# Autodesk Inventor assembly: lower arm full Assembly 800.ipt
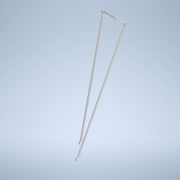
[picture p0: Inventor's stored thumbnail of the model, 180x180]
Saved by Autodesk Inventor 2021 (Build 250183000, 183)
## iProperties
Created: 2022-09-08
Part Number: lower arm full Assembly 800.ipt
Document SubType Name: Assembly
Designer: Administrator
Title: lower arm
Author: Administrator
## Documents named in this file (6)
- C:\Users\szucs\Desktop\GTPR\ver2\lower arm full Assembly 800.ipt.iam
- C:\Users\szucs\Desktop\GTPR\ver2\elbow keeper v1.ipt
- C:\Users\szucs\Desktop\GTPR\ver2\washer v1.ipt
- C:\Users\szucs\Desktop\GTPR\ver2\M8 Nut v5 v1.ipt
- C:\Users\szucs\Desktop\GTPR\ver2\lower arm Assembly 800.ipt.iam
- lower arm Assembly 800.ipt
## Components (13 placed, 4 different names)
1. elbow keeper v1:1 — Mate:1, Mate:3, Mate:6, Mate:7
2. washer v1:1 — Mate:2
3. washer v1:2 — Mate:9, Mate:10
4. washer v1:3 — Mate:8
5. washer v1:4 — Mate:4
6. M8 Nut v5 v1:1
7. M8 Nut v5 v1:2 — Flush:2
8. M8 Nut v5 v1:3 — Flush:1, Mate:10
9. M8 Nut v5 v1:4
10. lower arm Assembly 800.ipt:1 [sub-assembly] — Mate:1, Mate:2, Mate:9
11. lower arm Assembly 800.ipt:2 [sub-assembly] — Mate:3, Mate:4, Mate:8
12. M8 Nut v5 v1:5 — Flush:2, Mate:7
13. M8 Nut v5 v1:6 — Flush:1, Mate:6
## Relationships (11: Mate 9, Flush 2)
- Mate:1: elbow keeper v1:1 ↔ lower arm Assembly 800.ipt:1
- Mate:2: washer v1:1 ↔ lower arm Assembly 800.ipt:1
- Mate:3: elbow keeper v1:1 ↔ lower arm Assembly 800.ipt:2
- Mate:4: washer v1:4 ↔ lower arm Assembly 800.ipt:2
- Flush:1 (-22.5 mm): M8 Nut v5 v1:3 ↔ M8 Nut v5 v1:6
- Mate:6: elbow keeper v1:1 ↔ M8 Nut v5 v1:6
- Flush:2 (-22.5 mm): M8 Nut v5 v1:2 ↔ M8 Nut v5 v1:5
- Mate:7: elbow keeper v1:1 ↔ M8 Nut v5 v1:5
- Mate:8: washer v1:3 ↔ lower arm Assembly 800.ipt:2
- Mate:9: washer v1:2 ↔ lower arm Assembly 800.ipt:1
- Mate:10: washer v1:2 ↔ M8 Nut v5 v1:3
